# Autodesk Inventor assembly: mirror_with_magnets
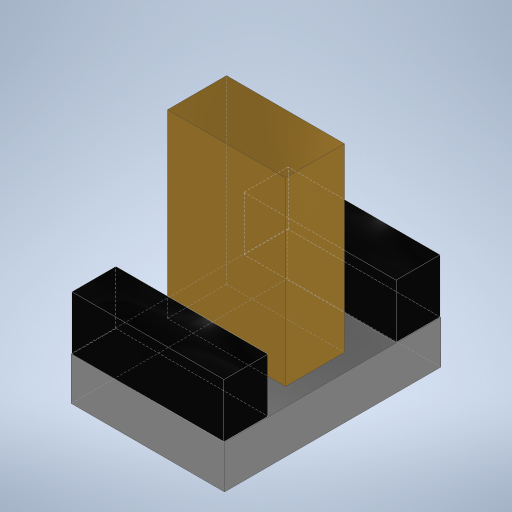
[picture p0: Inventor's stored thumbnail of the model, 512x512]
Saved by Autodesk Inventor 2023 (Build 270158000, 158)
## iProperties
Created: 2023-04-11
Part Number: mirror_with_magnets
Document SubType Name: Assembly
Designer: Sam
Author: Sam
## Documents named in this file (3)
- C:\Users\Sam\Desktop\Glasspin\mirror_with_magnets.iam
- C:\Users\Sam\Desktop\Glasspin\mirror.ipt
- C:\Users\Sam\Desktop\Glasspin\magnet.ipt
## Components (3 placed, 2 different names)
1. mirror:1 — Mate:2, Flush:4, Mate:4, Flush:5
2. magnet:1 — Mate:1, Mate:2, Flush:4
3. magnet:2 — Mate:3, Mate:4, Flush:5
## Relationships (6: Mate 4, Flush 2)
- Mate:1: magnet:1
- Mate:2: mirror:1 ↔ magnet:1
- Flush:4: mirror:1 ↔ magnet:1
- Mate:3: magnet:2
- Mate:4: mirror:1 ↔ magnet:2
- Flush:5: mirror:1 ↔ magnet:2
